# Autodesk Inventor assembly: Assembly - Whole - 9V base
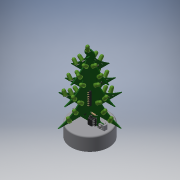
[picture p0: Inventor's stored thumbnail of the model, 180x180]
Saved by Autodesk Inventor 2018.3 (Build 223284000, 284)
## iProperties
Created: 2019-07-25
Part Number: Assembly - Whole - 9V base
Document SubType Name: Assembly
Designer: Electro707
Author: Electro707
## iProperties of the stored document 9V Battery.ipt
Created: 2017-10-09
Part Number: 9V Battery
Material: Generic
Description: STEP AP214
Document SubType Name: Modeling
Designer: Electro707
Density: 1 g/cm^3
Appearance: Default
Mass: 20.1787 g
Surface Area: 53.7975 cm^2
Volume: 20.1787 cm^3
Preprocessor: SwSTEP 2.0
Title: 9V Battery.STEP
Author: M.B.I.
Revision Number: ANY
## Documents named in this file (9)
- **F:\Projects\UNH MakerSpace Kits\2019 - Winter Holiday\Dual Tree Construction\CAD-Inventor\Assembly - Whole - 9V base.iam*LocalDocs*xSphvqfpvVh53eyg1TzwydrkyXe*9V Battery.ipt
- F:\Projects\UNH MakerSpace Kits\2019 - Winter Holiday\Dual Tree Construction\GitHub Folder\CAD - Inventor\Assembly - Whole - 9V base.iam
- C:\Users\Electro707\Documents\Inventor\Content Center Files\R2018\en-US\BS 4183(1)\BS 4183 - M3(1).ipt
- C:\Users\Electro707\Documents\Inventor\Content Center Files\R2018\en-US\ANSI B18.6.7M(00)\ANSI B18.6.7M - M3x0.5 x 8(4).ipt
- F:\Projects\UNH MakerSpace Kits\2019 - Winter Holiday\Dual Tree Construction\GitHub Folder\CAD - Inventor\Assembly - Main Tree.iam
- F:\Projects\UNH MakerSpace Kits\2019 - Winter Holiday\Dual Tree Construction\GitHub Folder\CAD - Inventor\Assembly - Aux Tree.iam
- F:\Projects\UNH MakerSpace Kits\2019 - Winter Holiday\Dual Tree Construction\GitHub Folder\CAD - Inventor\Base with 9V Batt.ipt
- **F:\Projects\UNH MakerSpace Kits\2019 - Winter Holiday\Dual Tree Construction\GitHub Folder\CAD - Inventor\Assembly - Whole - 9V base.iam*LocalDocs*xSphvqfpvVh53eyg1TzwydrkyXe*9V Battery.ipt
- F:\Projects\UNH MakerSpace Kits\2019 - Winter Holiday\Dual Tree Construction\GitHub Folder\CAD - Inventor\9V Battery.STEP
## Components (9 placed, 6 different names)
1. Cross Recessed Pan Head Machine Screw - Type I - Metric M3x0.5 x 8:1 — Mate:71, Mate:86
2. Cross Recessed Pan Head Machine Screw - Type I - Metric M3x0.5 x 8:2 — Mate:72, Mate:87
3. BS 4183 - Metric M3:3 — Mate:68
4. BS 4183 - Metric M3:4 — Mate:69, Mate:88
5. Assembly - Main Tree:1 [sub-assembly] — Mate:71, Mate:72, Mate:73, Mate:74, Cylindrical:1, Cylindrical:2, Cylindrical:3, Cylindrical:4, Mate:75, Mate:76, Mate:77, Mate:78
6. Assembly - Aux Tree:1 [sub-assembly] — Mate:73, Cylindrical:3, Cylindrical:4
7. Assembly - Aux Tree:2 [sub-assembly] — Mate:74, Cylindrical:1, Cylindrical:2
8. Base with 9V Batt:1 — Mate:75, Mate:76, Mate:79, Mate:80, Mate:82, Mate:83, Mate:85, Angle:2, Mate:86, Mate:87, Mate:88
9. 9V Battery:1 — Mate:82, Mate:83, Mate:84, Angle:1
## Relationships (30: Mate 23, CylindricalJoint 4, Angle 2, Flush 1)
- [Mate]: Cross Recessed Pan Head Machine Screw - Type I - Metric M3x0.5 x 8:2 ↔ BS 4183 - Metric M3:4
- [Mate]: Cross Recessed Pan Head Machine Screw - Type I - Metric M3x0.5 x 8:1 ↔ BS 4183 - Metric M3:3
- Mate:68: BS 4183 - Metric M3:3
- Mate:69: BS 4183 - Metric M3:4
- Mate:70
- Mate:71: Cross Recessed Pan Head Machine Screw - Type I - Metric M3x0.5 x 8:1 ↔ Assembly - Main Tree:1
- Mate:72: Cross Recessed Pan Head Machine Screw - Type I - Metric M3x0.5 x 8:2 ↔ Assembly - Main Tree:1
- Mate:73: Assembly - Main Tree:1 ↔ Assembly - Aux Tree:1
- Mate:74: Assembly - Main Tree:1 ↔ Assembly - Aux Tree:2
- Cylindrical:1: Assembly - Main Tree:1 ↔ Assembly - Aux Tree:2
- Cylindrical:2: Assembly - Main Tree:1 ↔ Assembly - Aux Tree:2
- Cylindrical:3: Assembly - Main Tree:1 ↔ Assembly - Aux Tree:1
- Cylindrical:4: Assembly - Main Tree:1 ↔ Assembly - Aux Tree:1
- Mate:75: Assembly - Main Tree:1 ↔ Base with 9V Batt:1
- Mate:76: Assembly - Main Tree:1 ↔ Base with 9V Batt:1
- Mate:77: Assembly - Main Tree:1
- Mate:78: Assembly - Main Tree:1
- Mate:79: Base with 9V Batt:1
- Mate:80: Base with 9V Batt:1
- Mate:81
- Mate:82: Base with 9V Batt:1 ↔ 9V Battery:1
- Mate:83: Base with 9V Batt:1 ↔ 9V Battery:1
- Mate:84: 9V Battery:1
- Angle:1 (0 deg): 9V Battery:1
- Mate:85: Base with 9V Batt:1
- Angle:2 (0 deg): Base with 9V Batt:1
- Flush:1
- Mate:86: Cross Recessed Pan Head Machine Screw - Type I - Metric M3x0.5 x 8:1 ↔ Base with 9V Batt:1
- Mate:87: Cross Recessed Pan Head Machine Screw - Type I - Metric M3x0.5 x 8:2 ↔ Base with 9V Batt:1
- Mate:88: BS 4183 - Metric M3:4 ↔ Base with 9V Batt:1
